# Autodesk Inventor assembly: Assembly1
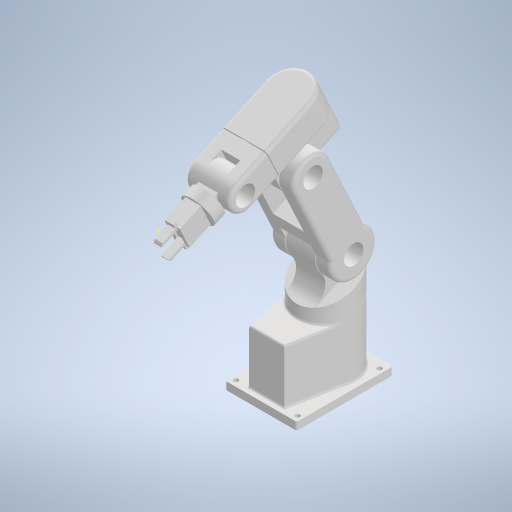
[picture p0: Inventor's stored thumbnail of the model, 512x512]
Saved by Autodesk Inventor 2024.1 (Build 281209000, 209)
## iProperties
Created: 2023-09-05
Part Number: Assembly1
Document SubType Name: Assembly
Designer: admins
Author: admins
## Documents named in this file (10)
- C:\Users\admins\Downloads\3D class\Assembly1.iam
- C:\Users\admins\Downloads\3D class\part1.ipt
- C:\Users\admins\Downloads\3D class\part2.ipt
- C:\Users\admins\Downloads\3D class\part4.ipt
- C:\Users\admins\Downloads\3D class\part6.ipt
- C:\Users\admins\Downloads\3D class\clamp.ipt
- C:\Users\admins\Downloads\3D class\mount.ipt
- C:\Users\admins\Downloads\3D class\part7.ipt
- C:\Users\admins\Downloads\3D class\part5.ipt
- C:\Users\admins\Downloads\3D class\part3.ipt
## Components (10 placed, 9 different names)
1. part1:1 — Rotational:1, Rotational:2
2. part2:1 — Rotational:2, Rotational:3
3. part4:1 — Rotational:4, Rotational:5
4. part6:1 — Rotational:6, Rotational:7
5. clamp:1 — Rigid:2
6. mount:1 — Rotational:7, Rigid:1, Rigid:2
7. part7:1 — Rotational:1
8. part5:1 — Rotational:5, Rotational:6
9. part3:1 — Rotational:3, Rotational:4
10. clamp:2 — Rigid:1
## Relationships (9: RevoluteJoint 7, WeldJoint 2)
- Rotational:1 [RevoluteJoint]: part1:1 ↔ part7:1
- Rotational:2 [RevoluteJoint]: part1:1 ↔ part2:1
- Rotational:3 [RevoluteJoint]: part2:1 ↔ part3:1
- Rotational:4 [RevoluteJoint]: part4:1 ↔ part3:1
- Rotational:5 [RevoluteJoint]: part4:1 ↔ part5:1
- Rotational:6 [RevoluteJoint]: part6:1 ↔ part5:1
- Rotational:7 [RevoluteJoint]: part6:1 ↔ mount:1
- Rigid:1 [WeldJoint]: mount:1 ↔ clamp:2
- Rigid:2 [WeldJoint]: clamp:1 ↔ mount:1
